# Autodesk Inventor assembly: 試作品2号
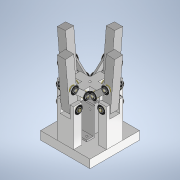
[picture p0: Inventor's stored thumbnail of the model, 180x180]
Saved by Autodesk Inventor 2021 (Build 250183000, 183)
## iProperties
Created: 2021-10-17
Part Number: 試作品2号
Document SubType Name: Assembly
Designer: ryusei
Author: ryusei
## Documents named in this file (15)
- C:\Users\ryusei\Documents\Inventor\robot_design3\試作品2号\試作品2号.iam
- C:\Users\ryusei\Documents\Inventor\robot_design3\試作品2号\部品\ハンド土台.ipt
- C:\Users\ryusei\Documents\Inventor\robot_design3\試作品2号\部品\ハンド支え.ipt
- C:\Users\ryusei\Documents\Inventor\robot_design3\試作品2号\部品\シリンダ固定.ipt
- C:\Users\ryusei\Documents\Inventor\robot_design3\試作品2号\部品\MBDA6×15_シリンダコガネイ\本体.ipt
- C:\Users\ryusei\Documents\Inventor\robot_design3\試作品2号\部品\MBDA6×15_シリンダコガネイ\伸びるやつ１.ipt
- C:\Users\ryusei\Documents\Inventor\robot_design3\試作品2号\部品\MBDA6×15_シリンダコガネイ\伸びるやつ2.ipt
- C:\Users\ryusei\Documents\Inventor\robot_design3\試作品2号\部品\シリンダ先端パーツ.ipt
- C:\Users\ryusei\Documents\Inventor\robot_design3\試作品2号\部品\MF63ZZ_ベアリング.ipt
- C:\Users\ryusei\Documents\Inventor\robot_design3\試作品2号\部品\Φ3軸用プッシュナット.ipt
- C:\Users\ryusei\Documents\Inventor\robot_design3\試作品2号\部品\ステンレス平行ピンΦ3h7_18.ipt
- C:\Users\ryusei\Documents\Inventor\robot_design3\試作品2号\部品\ステンレス平行ピンΦ3h7_25.ipt
- C:\Users\ryusei\Documents\Inventor\robot_design3\試作品2号\部品\樹脂ワッシャ(ポリスライダー).ipt
- C:\Users\ryusei\Documents\Inventor\robot_design3\試作品2号\部品\ハンド10×10×60.ipt
- C:\Users\ryusei\Documents\Inventor\robot_design3\試作品2号\部品\リンク26×6×2.ipt
## Components (147 placed, 14 different names)
1. ハンド土台:1 — 挿入:1, 挿入:2, 挿入:3, 挿入:4, 挿入:5, 挿入:6, 挿入:7, 挿入:8, 挿入:9, 挿入:10, 挿入:11, 挿入:12
2. ハンド支え:1 — 挿入:1, 挿入:2, 挿入:21, 挿入:22, 挿入:151, 挿入:153
3. ハンド支え:2 — 挿入:3, 挿入:4, 挿入:19, 挿入:20, 挿入:147, 挿入:149
4. ハンド支え:3 — 挿入:5, 挿入:6, 挿入:25, 挿入:26, 挿入:159, 挿入:161
5. ハンド支え:4 — 挿入:7, 挿入:8, 角度:1, 挿入:23, 挿入:24, 挿入:155, 挿入:157
6. シリンダ固定:1 — 挿入:11, 挿入:12, 挿入:13, 挿入:14
7. シリンダ固定:2 — 挿入:9, 挿入:10, 挿入:15, 挿入:16
8. 本体:1 — 挿入:13, 挿入:14, 挿入:15, 挿入:16, メイト:1, 円柱状:1
9. 伸びるやつ１:1 — 挿入:17, メイト:1, 円柱状:1
10. 伸びるやつ2:1 — 挿入:17, 挿入:18
11. シリンダ先端パーツ:2 — 挿入:18, 角度:1, 挿入:27, 挿入:28, 挿入:29, 挿入:30, 挿入:31, 挿入:32, 挿入:33, 挿入:34
12. MF63ZZ_ベアリング:1 — 挿入:21, 挿入:45
13. MF63ZZ_ベアリング:2 — 挿入:23, 挿入:40, 挿入:49
14. MF63ZZ_ベアリング:3 — 挿入:22, 挿入:41, 挿入:43
15. MF63ZZ_ベアリング:4 — 挿入:27, 挿入:85
16. MF63ZZ_ベアリング:5 — 挿入:19, 挿入:53
17. MF63ZZ_ベアリング:6 — 挿入:28, 挿入:38, 挿入:89
18. MF63ZZ_ベアリング:7 — 挿入:24, 挿入:57
19. MF63ZZ_ベアリング:8 — 挿入:30, 挿入:86
20. MF63ZZ_ベアリング:9 — 挿入:25, 挿入:51
21. MF63ZZ_ベアリング:10 — 挿入:32, 挿入:35, 挿入:96
22. MF63ZZ_ベアリング:11 — 挿入:34, 挿入:98
23. MF63ZZ_ベアリング:12 — 挿入:33, 挿入:36, 挿入:95
24. MF63ZZ_ベアリング:13 — 挿入:31, 挿入:37, 挿入:93
25. MF63ZZ_ベアリング:14 — 挿入:29, 挿入:91
26. MF63ZZ_ベアリング:15 — 挿入:26, 挿入:39, 挿入:55
27. MF63ZZ_ベアリング:16 — 挿入:20, 挿入:42, 挿入:47
28. ステンレス平行ピンΦ3h7_18:1 — 挿入:36
29. ステンレス平行ピンΦ3h7_18:2 — 挿入:37
30. ステンレス平行ピンΦ3h7_18:3 — 挿入:38
31. ステンレス平行ピンΦ3h7_18:4 — 挿入:35
32. ステンレス平行ピンΦ3h7_25:1 — 挿入:39, 挿入:70
33. ステンレス平行ピンΦ3h7_25:2 — 挿入:40, 挿入:69
34. ステンレス平行ピンΦ3h7_25:3 — 挿入:41, 挿入:67
35. ステンレス平行ピンΦ3h7_25:4 — 挿入:42, 挿入:68
36. 樹脂ワッシャ(ポリスライダー):1 — 挿入:49, 挿入:50
37. 樹脂ワッシャ(ポリスライダー):2 — 挿入:54, 挿入:60
38. 樹脂ワッシャ(ポリスライダー):3 — 挿入:50, 挿入:63
39. 樹脂ワッシャ(ポリスライダー):4 — 挿入:46, 挿入:61
40. 樹脂ワッシャ(ポリスライダー):5 — 挿入:52, 挿入:66
41. 樹脂ワッシャ(ポリスライダー):6 — 挿入:58, 挿入:65
42. 樹脂ワッシャ(ポリスライダー):7 — 挿入:55, 挿入:56
43. 樹脂ワッシャ(ポリスライダー):8 — 挿入:57, 挿入:58
44. 樹脂ワッシャ(ポリスライダー):9 — 挿入:53, 挿入:54
45. 樹脂ワッシャ(ポリスライダー):10 — 挿入:44, 挿入:62
46. 樹脂ワッシャ(ポリスライダー):11 — 挿入:56, 挿入:64
47. 樹脂ワッシャ(ポリスライダー):12 — 挿入:51, 挿入:52
48. 樹脂ワッシャ(ポリスライダー):13 — 挿入:48, 挿入:59
49. 樹脂ワッシャ(ポリスライダー):14 — 挿入:47, 挿入:48
50. 樹脂ワッシャ(ポリスライダー):15 — 挿入:43, 挿入:44
51. 樹脂ワッシャ(ポリスライダー):16 — 挿入:45, 挿入:46
52. Φ3軸用プッシュナット:1 — 挿入:60
53. Φ3軸用プッシュナット:2 — 挿入:61
54. Φ3軸用プッシュナット:3 — 挿入:62
55. Φ3軸用プッシュナット:4 — 挿入:59
56. Φ3軸用プッシュナット:5 — 挿入:66
57. Φ3軸用プッシュナット:6 — 挿入:63
58. Φ3軸用プッシュナット:7 — 挿入:65
59. Φ3軸用プッシュナット:8 — 挿入:64
60. ハンド10×10×60:1 — 挿入:69, 挿入:74, 挿入:78
61. ハンド10×10×60:2 — 挿入:67, 挿入:73, 挿入:76
62. ハンド10×10×60:3 — 挿入:70, 挿入:71, 挿入:75
63. ハンド10×10×60:4 — 挿入:68, 挿入:72, 挿入:77
64. MF63ZZ_ベアリング:17 — 挿入:76, 挿入:92
65. MF63ZZ_ベアリング:18 — 挿入:73, 挿入:82, 挿入:90
66. MF63ZZ_ベアリング:19 — 挿入:74, 挿入:80, 挿入:97
67. MF63ZZ_ベアリング:20 — 挿入:72, 挿入:81, 挿入:83
68. MF63ZZ_ベアリング:21 — 挿入:71, 挿入:79, 挿入:87
69. MF63ZZ_ベアリング:22 — 挿入:75, 挿入:84
70. MF63ZZ_ベアリング:23 — 挿入:78, 挿入:94
71. MF63ZZ_ベアリング:24 — 挿入:77, 挿入:88
72. ステンレス平行ピンΦ3h7_18:5 — 挿入:81
73. ステンレス平行ピンΦ3h7_18:6 — 挿入:82
74. ステンレス平行ピンΦ3h7_18:7 — 挿入:79
75. ステンレス平行ピンΦ3h7_18:8 — 挿入:80
76. 樹脂ワッシャ(ポリスライダー):17 — 挿入:96, 挿入:101
77. 樹脂ワッシャ(ポリスライダー):18 — 挿入:87, 挿入:100
78. 樹脂ワッシャ(ポリスライダー):19 — 挿入:97, 挿入:104
79. 樹脂ワッシャ(ポリスライダー):20 — 挿入:89, 挿入:112
80. 樹脂ワッシャ(ポリスライダー):21 — 挿入:95, 挿入:107
81. 樹脂ワッシャ(ポリスライダー):22 — 挿入:88, 挿入:111
82. 樹脂ワッシャ(ポリスライダー):23 — 挿入:93, 挿入:106
83. 樹脂ワッシャ(ポリスライダー):24 — 挿入:90, 挿入:109
84. 樹脂ワッシャ(ポリスライダー):25 — 挿入:92, 挿入:105
85. 樹脂ワッシャ(ポリスライダー):26 — 挿入:94, 挿入:108
86. 樹脂ワッシャ(ポリスライダー):27 — 挿入:91, 挿入:110
87. 樹脂ワッシャ(ポリスライダー):28 — 挿入:85, 挿入:113
88. 樹脂ワッシャ(ポリスライダー):29 — 挿入:83, 挿入:114
89. 樹脂ワッシャ(ポリスライダー):30 — 挿入:84, 挿入:102
90. 樹脂ワッシャ(ポリスライダー):31 — 挿入:86, 挿入:99
91. 樹脂ワッシャ(ポリスライダー):32 — 挿入:98, 挿入:103
92. リンク26×6×2:1 — 挿入:105, 挿入:106, 挿入:128, 挿入:129
93. リンク26×6×2:2 — 挿入:103, 挿入:104, 挿入:125, 挿入:130
94. リンク26×6×2:3 — 挿入:101, 挿入:102, 挿入:123, 挿入:124
95. リンク26×6×2:4 — 挿入:99, 挿入:100, 挿入:117, 挿入:118
96. リンク26×6×2:5 — 挿入:107, 挿入:108, 挿入:126, 挿入:127
97. リンク26×6×2:6 — 挿入:109, 挿入:110, 挿入:121, 挿入:122
98. リンク26×6×2:7 — 挿入:111, 挿入:112, 挿入:119, 挿入:120
99. リンク26×6×2:8 — 挿入:113, 挿入:114, 挿入:115, 挿入:116
100. 樹脂ワッシャ(ポリスライダー):33 — 挿入:122, 挿入:142
101. 樹脂ワッシャ(ポリスライダー):34 — 挿入:117, 挿入:131
102. 樹脂ワッシャ(ポリスライダー):35 — 挿入:119, 挿入:143
103. 樹脂ワッシャ(ポリスライダー):36 — 挿入:115, 挿入:145
104. 樹脂ワッシャ(ポリスライダー):37 — 挿入:120, 挿入:144
105. 樹脂ワッシャ(ポリスライダー):38 — 挿入:121, 挿入:141
106. 樹脂ワッシャ(ポリスライダー):39 — 挿入:118, 挿入:132
107. 樹脂ワッシャ(ポリスライダー):40 — 挿入:116, 挿入:146
108. 樹脂ワッシャ(ポリスライダー):41 — 挿入:125, 挿入:136
109. 樹脂ワッシャ(ポリスライダー):42 — 挿入:126, 挿入:137
110. 樹脂ワッシャ(ポリスライダー):43 — 挿入:128, 挿入:140
111. 樹脂ワッシャ(ポリスライダー):44 — 挿入:123, 挿入:134
112. 樹脂ワッシャ(ポリスライダー):45 — 挿入:129, 挿入:139
113. 樹脂ワッシャ(ポリスライダー):46 — 挿入:124, 挿入:133
114. 樹脂ワッシャ(ポリスライダー):47 — 挿入:127, 挿入:138
115. 樹脂ワッシャ(ポリスライダー):48 — 挿入:130, 挿入:135
116. Φ3軸用プッシュナット:9 — 挿入:136
117. Φ3軸用プッシュナット:10 — 挿入:135
118. Φ3軸用プッシュナット:11 — 挿入:137
119. Φ3軸用プッシュナット:12 — 挿入:138
120. Φ3軸用プッシュナット:13 — 挿入:131
121. Φ3軸用プッシュナット:14 — 挿入:134
122. Φ3軸用プッシュナット:15 — 挿入:132
123. Φ3軸用プッシュナット:16 — 挿入:133
124. Φ3軸用プッシュナット:17 — 挿入:139
125. Φ3軸用プッシュナット:18 — 挿入:140
126. Φ3軸用プッシュナット:19 — 挿入:142
127. Φ3軸用プッシュナット:20 — 挿入:141
128. Φ3軸用プッシュナット:21 — 挿入:143
129. Φ3軸用プッシュナット:22 — 挿入:144
130. Φ3軸用プッシュナット:23 — 挿入:145
131. Φ3軸用プッシュナット:24 — 挿入:146
132. 樹脂ワッシャ(ポリスライダー):49 — 挿入:151, 挿入:152
133. 樹脂ワッシャ(ポリスライダー):50 — 挿入:149, 挿入:150
134. 樹脂ワッシャ(ポリスライダー):51 — 挿入:148
135. 樹脂ワッシャ(ポリスライダー):52 — 挿入:152
136. 樹脂ワッシャ(ポリスライダー):53 — 挿入:153, 挿入:154
137. 樹脂ワッシャ(ポリスライダー):54 — 挿入:154
138. 樹脂ワッシャ(ポリスライダー):55 — 挿入:150
139. 樹脂ワッシャ(ポリスライダー):56 — 挿入:147, 挿入:148
140. 樹脂ワッシャ(ポリスライダー):57 — 挿入:156
141. 樹脂ワッシャ(ポリスライダー):58 — 挿入:157, 挿入:158
142. 樹脂ワッシャ(ポリスライダー):59 — 挿入:158
143. 樹脂ワッシャ(ポリスライダー):60 — 挿入:155, 挿入:156
144. 樹脂ワッシャ(ポリスライダー):61 — 挿入:160
145. 樹脂ワッシャ(ポリスライダー):62 — 挿入:159, 挿入:160
146. 樹脂ワッシャ(ポリスライダー):63 — 挿入:161, 挿入:162
147. 樹脂ワッシャ(ポリスライダー):64 — 挿入:162
## Relationships (165: Insert 162, Mate 1, CylindricalJoint 1, Angle 1)
- 挿入:1 [Insert]: ハンド土台:1 ↔ ハンド支え:1
- 挿入:2 [Insert]: ハンド土台:1 ↔ ハンド支え:1
- 挿入:3 [Insert]: ハンド土台:1 ↔ ハンド支え:2
- 挿入:4 [Insert]: ハンド土台:1 ↔ ハンド支え:2
- 挿入:5 [Insert]: ハンド土台:1 ↔ ハンド支え:3
- 挿入:6 [Insert]: ハンド土台:1 ↔ ハンド支え:3
- 挿入:7 [Insert]: ハンド土台:1 ↔ ハンド支え:4
- 挿入:8 [Insert]: ハンド土台:1 ↔ ハンド支え:4
- 挿入:9 [Insert]: ハンド土台:1 ↔ シリンダ固定:2
- 挿入:10 [Insert]: ハンド土台:1 ↔ シリンダ固定:2
- 挿入:11 [Insert]: ハンド土台:1 ↔ シリンダ固定:1
- 挿入:12 [Insert]: ハンド土台:1 ↔ シリンダ固定:1
- 挿入:13 [Insert]: シリンダ固定:1 ↔ 本体:1
- 挿入:14 [Insert]: シリンダ固定:1 ↔ 本体:1
- 挿入:15 [Insert]: シリンダ固定:2 ↔ 本体:1
- 挿入:16 [Insert]: シリンダ固定:2 ↔ 本体:1
- 挿入:17 [Insert]: 伸びるやつ１:1 ↔ 伸びるやつ2:1
- メイト:1 [Mate]: 本体:1 ↔ 伸びるやつ１:1
- 円柱状:1 [CylindricalJoint]: 本体:1 ↔ 伸びるやつ１:1
- 挿入:18 [Insert]: 伸びるやつ2:1 ↔ シリンダ先端パーツ:2
- 角度:1 [Angle] (0 deg): ハンド支え:4 ↔ シリンダ先端パーツ:2
- 挿入:19 [Insert]: ハンド支え:2 ↔ MF63ZZ_ベアリング:5
- 挿入:20 [Insert]: ハンド支え:2 ↔ MF63ZZ_ベアリング:16
- 挿入:21 [Insert]: ハンド支え:1 ↔ MF63ZZ_ベアリング:1
- 挿入:22 [Insert]: ハンド支え:1 ↔ MF63ZZ_ベアリング:3
- 挿入:23 [Insert]: ハンド支え:4 ↔ MF63ZZ_ベアリング:2
- 挿入:24 [Insert]: ハンド支え:4 ↔ MF63ZZ_ベアリング:7
- 挿入:25 [Insert]: ハンド支え:3 ↔ MF63ZZ_ベアリング:9
- 挿入:26 [Insert]: ハンド支え:3 ↔ MF63ZZ_ベアリング:15
- 挿入:27 [Insert]: シリンダ先端パーツ:2 ↔ MF63ZZ_ベアリング:4
- 挿入:28 [Insert]: シリンダ先端パーツ:2 ↔ MF63ZZ_ベアリング:6
- 挿入:29 [Insert]: シリンダ先端パーツ:2 ↔ MF63ZZ_ベアリング:14
- 挿入:30 [Insert]: シリンダ先端パーツ:2 ↔ MF63ZZ_ベアリング:8
- 挿入:31 [Insert]: シリンダ先端パーツ:2 ↔ MF63ZZ_ベアリング:13
- 挿入:32 [Insert]: シリンダ先端パーツ:2 ↔ MF63ZZ_ベアリング:10
- 挿入:33 [Insert]: シリンダ先端パーツ:2 ↔ MF63ZZ_ベアリング:12
- 挿入:34 [Insert]: シリンダ先端パーツ:2 ↔ MF63ZZ_ベアリング:11
- 挿入:35 [Insert] (-3.4 mm): MF63ZZ_ベアリング:10 ↔ ステンレス平行ピンΦ3h7_18:4
- 挿入:36 [Insert] (-3.4 mm): MF63ZZ_ベアリング:12 ↔ ステンレス平行ピンΦ3h7_18:1
- 挿入:37 [Insert] (-3.4 mm): MF63ZZ_ベアリング:13 ↔ ステンレス平行ピンΦ3h7_18:2
- 挿入:38 [Insert] (-3.4 mm): MF63ZZ_ベアリング:6 ↔ ステンレス平行ピンΦ3h7_18:3
- 挿入:39 [Insert] (-1.9 mm): MF63ZZ_ベアリング:15 ↔ ステンレス平行ピンΦ3h7_25:1
- 挿入:40 [Insert] (-1.9 mm): MF63ZZ_ベアリング:2 ↔ ステンレス平行ピンΦ3h7_25:2
- 挿入:41 [Insert] (-1.9 mm): MF63ZZ_ベアリング:3 ↔ ステンレス平行ピンΦ3h7_25:3
- 挿入:42 [Insert] (-1.9 mm): MF63ZZ_ベアリング:16 ↔ ステンレス平行ピンΦ3h7_25:4
- 挿入:43 [Insert]: MF63ZZ_ベアリング:3 ↔ 樹脂ワッシャ(ポリスライダー):15
- 挿入:44 [Insert]: 樹脂ワッシャ(ポリスライダー):10 ↔ 樹脂ワッシャ(ポリスライダー):15
- 挿入:45 [Insert]: MF63ZZ_ベアリング:1 ↔ 樹脂ワッシャ(ポリスライダー):16
- 挿入:46 [Insert]: 樹脂ワッシャ(ポリスライダー):4 ↔ 樹脂ワッシャ(ポリスライダー):16
- 挿入:47 [Insert]: MF63ZZ_ベアリング:16 ↔ 樹脂ワッシャ(ポリスライダー):14
- 挿入:48 [Insert]: 樹脂ワッシャ(ポリスライダー):13 ↔ 樹脂ワッシャ(ポリスライダー):14
- 挿入:49 [Insert]: MF63ZZ_ベアリング:2 ↔ 樹脂ワッシャ(ポリスライダー):1
- 挿入:50 [Insert]: 樹脂ワッシャ(ポリスライダー):1 ↔ 樹脂ワッシャ(ポリスライダー):3
- 挿入:51 [Insert]: MF63ZZ_ベアリング:9 ↔ 樹脂ワッシャ(ポリスライダー):12
- 挿入:52 [Insert]: 樹脂ワッシャ(ポリスライダー):5 ↔ 樹脂ワッシャ(ポリスライダー):12
- 挿入:53 [Insert]: MF63ZZ_ベアリング:5 ↔ 樹脂ワッシャ(ポリスライダー):9
- 挿入:54 [Insert]: 樹脂ワッシャ(ポリスライダー):2 ↔ 樹脂ワッシャ(ポリスライダー):9
- 挿入:55 [Insert]: MF63ZZ_ベアリング:15 ↔ 樹脂ワッシャ(ポリスライダー):7
- 挿入:56 [Insert]: 樹脂ワッシャ(ポリスライダー):7 ↔ 樹脂ワッシャ(ポリスライダー):11
- 挿入:57 [Insert]: MF63ZZ_ベアリング:7 ↔ 樹脂ワッシャ(ポリスライダー):8
- 挿入:58 [Insert]: 樹脂ワッシャ(ポリスライダー):6 ↔ 樹脂ワッシャ(ポリスライダー):8
- 挿入:59 [Insert]: 樹脂ワッシャ(ポリスライダー):13 ↔ Φ3軸用プッシュナット:4
- 挿入:60 [Insert]: 樹脂ワッシャ(ポリスライダー):2 ↔ Φ3軸用プッシュナット:1
- 挿入:61 [Insert]: 樹脂ワッシャ(ポリスライダー):4 ↔ Φ3軸用プッシュナット:2
- 挿入:62 [Insert]: 樹脂ワッシャ(ポリスライダー):10 ↔ Φ3軸用プッシュナット:3
- 挿入:63 [Insert]: 樹脂ワッシャ(ポリスライダー):3 ↔ Φ3軸用プッシュナット:6
- 挿入:64 [Insert]: 樹脂ワッシャ(ポリスライダー):11 ↔ Φ3軸用プッシュナット:8
- 挿入:65 [Insert]: 樹脂ワッシャ(ポリスライダー):6 ↔ Φ3軸用プッシュナット:7
- 挿入:66 [Insert]: 樹脂ワッシャ(ポリスライダー):5 ↔ Φ3軸用プッシュナット:5
- 挿入:67 [Insert] (-7.5 mm): ステンレス平行ピンΦ3h7_25:3 ↔ ハンド10×10×60:2
- 挿入:68 [Insert] (-7.5 mm): ステンレス平行ピンΦ3h7_25:4 ↔ ハンド10×10×60:4
- 挿入:69 [Insert] (-7.5 mm): ステンレス平行ピンΦ3h7_25:2 ↔ ハンド10×10×60:1
- 挿入:70 [Insert] (-7.5 mm): ステンレス平行ピンΦ3h7_25:1 ↔ ハンド10×10×60:3
- 挿入:71 [Insert]: ハンド10×10×60:3 ↔ MF63ZZ_ベアリング:21
- 挿入:72 [Insert]: ハンド10×10×60:4 ↔ MF63ZZ_ベアリング:20
- 挿入:73 [Insert]: ハンド10×10×60:2 ↔ MF63ZZ_ベアリング:18
- 挿入:74 [Insert]: ハンド10×10×60:1 ↔ MF63ZZ_ベアリング:19
- 挿入:75 [Insert]: ハンド10×10×60:3 ↔ MF63ZZ_ベアリング:22
- 挿入:76 [Insert]: ハンド10×10×60:2 ↔ MF63ZZ_ベアリング:17
- 挿入:77 [Insert]: ハンド10×10×60:4 ↔ MF63ZZ_ベアリング:24
- 挿入:78 [Insert]: ハンド10×10×60:1 ↔ MF63ZZ_ベアリング:23
- 挿入:79 [Insert] (-3.4 mm): MF63ZZ_ベアリング:21 ↔ ステンレス平行ピンΦ3h7_18:7
- 挿入:80 [Insert] (-3.4 mm): MF63ZZ_ベアリング:19 ↔ ステンレス平行ピンΦ3h7_18:8
- 挿入:81 [Insert] (-3.4 mm): MF63ZZ_ベアリング:20 ↔ ステンレス平行ピンΦ3h7_18:5
- 挿入:82 [Insert] (-3.4 mm): MF63ZZ_ベアリング:18 ↔ ステンレス平行ピンΦ3h7_18:6
- 挿入:83 [Insert]: MF63ZZ_ベアリング:20 ↔ 樹脂ワッシャ(ポリスライダー):29
- 挿入:84 [Insert]: MF63ZZ_ベアリング:22 ↔ 樹脂ワッシャ(ポリスライダー):30
- 挿入:85 [Insert]: MF63ZZ_ベアリング:4 ↔ 樹脂ワッシャ(ポリスライダー):28
- 挿入:86 [Insert]: MF63ZZ_ベアリング:8 ↔ 樹脂ワッシャ(ポリスライダー):31
- 挿入:87 [Insert]: MF63ZZ_ベアリング:21 ↔ 樹脂ワッシャ(ポリスライダー):18
- 挿入:88 [Insert]: MF63ZZ_ベアリング:24 ↔ 樹脂ワッシャ(ポリスライダー):22
- 挿入:89 [Insert]: MF63ZZ_ベアリング:6 ↔ 樹脂ワッシャ(ポリスライダー):20
- 挿入:90 [Insert]: MF63ZZ_ベアリング:18 ↔ 樹脂ワッシャ(ポリスライダー):24
- 挿入:91 [Insert]: MF63ZZ_ベアリング:14 ↔ 樹脂ワッシャ(ポリスライダー):27
- 挿入:92 [Insert]: MF63ZZ_ベアリング:17 ↔ 樹脂ワッシャ(ポリスライダー):25
- 挿入:93 [Insert]: MF63ZZ_ベアリング:13 ↔ 樹脂ワッシャ(ポリスライダー):23
- 挿入:94 [Insert]: MF63ZZ_ベアリング:23 ↔ 樹脂ワッシャ(ポリスライダー):26
- 挿入:95 [Insert]: MF63ZZ_ベアリング:12 ↔ 樹脂ワッシャ(ポリスライダー):21
- 挿入:96 [Insert]: MF63ZZ_ベアリング:10 ↔ 樹脂ワッシャ(ポリスライダー):17
- 挿入:97 [Insert]: MF63ZZ_ベアリング:19 ↔ 樹脂ワッシャ(ポリスライダー):19
- 挿入:98 [Insert]: MF63ZZ_ベアリング:11 ↔ 樹脂ワッシャ(ポリスライダー):32
- 挿入:99 [Insert]: 樹脂ワッシャ(ポリスライダー):31 ↔ リンク26×6×2:4
- 挿入:100 [Insert]: 樹脂ワッシャ(ポリスライダー):18 ↔ リンク26×6×2:4
- 挿入:101 [Insert]: 樹脂ワッシャ(ポリスライダー):17 ↔ リンク26×6×2:3
- 挿入:102 [Insert]: 樹脂ワッシャ(ポリスライダー):30 ↔ リンク26×6×2:3
- 挿入:103 [Insert]: 樹脂ワッシャ(ポリスライダー):32 ↔ リンク26×6×2:2
- 挿入:104 [Insert]: 樹脂ワッシャ(ポリスライダー):19 ↔ リンク26×6×2:2
- 挿入:105 [Insert]: 樹脂ワッシャ(ポリスライダー):25 ↔ リンク26×6×2:1
- 挿入:106 [Insert]: 樹脂ワッシャ(ポリスライダー):23 ↔ リンク26×6×2:1
- 挿入:107 [Insert]: 樹脂ワッシャ(ポリスライダー):21 ↔ リンク26×6×2:5
- 挿入:108 [Insert]: 樹脂ワッシャ(ポリスライダー):26 ↔ リンク26×6×2:5
- 挿入:109 [Insert]: 樹脂ワッシャ(ポリスライダー):24 ↔ リンク26×6×2:6
- 挿入:110 [Insert]: 樹脂ワッシャ(ポリスライダー):27 ↔ リンク26×6×2:6
- 挿入:111 [Insert]: 樹脂ワッシャ(ポリスライダー):22 ↔ リンク26×6×2:7
- 挿入:112 [Insert]: 樹脂ワッシャ(ポリスライダー):20 ↔ リンク26×6×2:7
- 挿入:113 [Insert]: 樹脂ワッシャ(ポリスライダー):28 ↔ リンク26×6×2:8
- 挿入:114 [Insert]: 樹脂ワッシャ(ポリスライダー):29 ↔ リンク26×6×2:8
- 挿入:115 [Insert]: リンク26×6×2:8 ↔ 樹脂ワッシャ(ポリスライダー):36
- 挿入:116 [Insert]: リンク26×6×2:8 ↔ 樹脂ワッシャ(ポリスライダー):40
- 挿入:117 [Insert]: リンク26×6×2:4 ↔ 樹脂ワッシャ(ポリスライダー):34
- 挿入:118 [Insert]: リンク26×6×2:4 ↔ 樹脂ワッシャ(ポリスライダー):39
- 挿入:119 [Insert]: リンク26×6×2:7 ↔ 樹脂ワッシャ(ポリスライダー):35
- 挿入:120 [Insert]: リンク26×6×2:7 ↔ 樹脂ワッシャ(ポリスライダー):37
- 挿入:121 [Insert]: リンク26×6×2:6 ↔ 樹脂ワッシャ(ポリスライダー):38
- 挿入:122 [Insert]: リンク26×6×2:6 ↔ 樹脂ワッシャ(ポリスライダー):33
- 挿入:123 [Insert]: リンク26×6×2:3 ↔ 樹脂ワッシャ(ポリスライダー):44
- 挿入:124 [Insert]: リンク26×6×2:3 ↔ 樹脂ワッシャ(ポリスライダー):46
- 挿入:125 [Insert]: リンク26×6×2:2 ↔ 樹脂ワッシャ(ポリスライダー):41
- 挿入:126 [Insert]: リンク26×6×2:5 ↔ 樹脂ワッシャ(ポリスライダー):42
- 挿入:127 [Insert]: リンク26×6×2:5 ↔ 樹脂ワッシャ(ポリスライダー):47
- 挿入:128 [Insert]: リンク26×6×2:1 ↔ 樹脂ワッシャ(ポリスライダー):43
- 挿入:129 [Insert]: リンク26×6×2:1 ↔ 樹脂ワッシャ(ポリスライダー):45
- 挿入:130 [Insert]: リンク26×6×2:2 ↔ 樹脂ワッシャ(ポリスライダー):48
- 挿入:131 [Insert]: 樹脂ワッシャ(ポリスライダー):34 ↔ Φ3軸用プッシュナット:13
- 挿入:132 [Insert]: 樹脂ワッシャ(ポリスライダー):39 ↔ Φ3軸用プッシュナット:15
- 挿入:133 [Insert]: 樹脂ワッシャ(ポリスライダー):46 ↔ Φ3軸用プッシュナット:16
- 挿入:134 [Insert]: 樹脂ワッシャ(ポリスライダー):44 ↔ Φ3軸用プッシュナット:14
- 挿入:135 [Insert]: 樹脂ワッシャ(ポリスライダー):48 ↔ Φ3軸用プッシュナット:10
- 挿入:136 [Insert]: 樹脂ワッシャ(ポリスライダー):41 ↔ Φ3軸用プッシュナット:9
- 挿入:137 [Insert]: 樹脂ワッシャ(ポリスライダー):42 ↔ Φ3軸用プッシュナット:11
- 挿入:138 [Insert]: 樹脂ワッシャ(ポリスライダー):47 ↔ Φ3軸用プッシュナット:12
- 挿入:139 [Insert]: 樹脂ワッシャ(ポリスライダー):45 ↔ Φ3軸用プッシュナット:17
- 挿入:140 [Insert]: 樹脂ワッシャ(ポリスライダー):43 ↔ Φ3軸用プッシュナット:18
- 挿入:141 [Insert]: 樹脂ワッシャ(ポリスライダー):38 ↔ Φ3軸用プッシュナット:20
- 挿入:142 [Insert]: 樹脂ワッシャ(ポリスライダー):33 ↔ Φ3軸用プッシュナット:19
- 挿入:143 [Insert]: 樹脂ワッシャ(ポリスライダー):35 ↔ Φ3軸用プッシュナット:21
- 挿入:144 [Insert]: 樹脂ワッシャ(ポリスライダー):37 ↔ Φ3軸用プッシュナット:22
- 挿入:145 [Insert]: 樹脂ワッシャ(ポリスライダー):36 ↔ Φ3軸用プッシュナット:23
- 挿入:146 [Insert]: 樹脂ワッシャ(ポリスライダー):40 ↔ Φ3軸用プッシュナット:24
- 挿入:147 [Insert]: ハンド支え:2 ↔ 樹脂ワッシャ(ポリスライダー):56
- 挿入:148 [Insert]: 樹脂ワッシャ(ポリスライダー):51 ↔ 樹脂ワッシャ(ポリスライダー):56
- 挿入:149 [Insert]: ハンド支え:2 ↔ 樹脂ワッシャ(ポリスライダー):50
- 挿入:150 [Insert]: 樹脂ワッシャ(ポリスライダー):50 ↔ 樹脂ワッシャ(ポリスライダー):55
- 挿入:151 [Insert]: ハンド支え:1 ↔ 樹脂ワッシャ(ポリスライダー):49
- 挿入:152 [Insert]: 樹脂ワッシャ(ポリスライダー):49 ↔ 樹脂ワッシャ(ポリスライダー):52
- 挿入:153 [Insert]: ハンド支え:1 ↔ 樹脂ワッシャ(ポリスライダー):53
- 挿入:154 [Insert]: 樹脂ワッシャ(ポリスライダー):53 ↔ 樹脂ワッシャ(ポリスライダー):54
- 挿入:155 [Insert]: ハンド支え:4 ↔ 樹脂ワッシャ(ポリスライダー):60
- 挿入:156 [Insert]: 樹脂ワッシャ(ポリスライダー):57 ↔ 樹脂ワッシャ(ポリスライダー):60
- 挿入:157 [Insert]: ハンド支え:4 ↔ 樹脂ワッシャ(ポリスライダー):58
- 挿入:158 [Insert]: 樹脂ワッシャ(ポリスライダー):58 ↔ 樹脂ワッシャ(ポリスライダー):59
- 挿入:159 [Insert]: ハンド支え:3 ↔ 樹脂ワッシャ(ポリスライダー):62
- 挿入:160 [Insert]: 樹脂ワッシャ(ポリスライダー):61 ↔ 樹脂ワッシャ(ポリスライダー):62
- 挿入:161 [Insert]: ハンド支え:3 ↔ 樹脂ワッシャ(ポリスライダー):63
- 挿入:162 [Insert]: 樹脂ワッシャ(ポリスライダー):63 ↔ 樹脂ワッシャ(ポリスライダー):64
